# Autodesk Inventor assembly: Bucket+Magnets
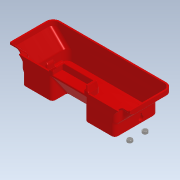
[picture p0: Inventor's stored thumbnail of the model, 180x180]
Saved by Autodesk Inventor 2022.1 (Build 261234020, 234B)
## iProperties
Created: 2022-07-24
Part Number: Bucket+Magnets
Document SubType Name: Assembly
Designer: Rama
Author: Rama
## Documents named in this file (3)
- C:\Users\Rama\Desktop\GitHub\Voron-2-Mods\Mandalaroseworks\BedPan\CAD\SRC\Manual_Helpers\Bucket+Magnets.iam
- C:\Users\Rama\Desktop\GitHub\Voron-2-Mods\Mandalaroseworks\BedPan\CAD\SRC\Bucket\Bucket_Offset.iam
- C:\Users\Rama\Desktop\RAMA_SBNG\ToolheadNEW\6x3 Magnet.ipt
## Components (5 placed, 2 different names)
1. Bucket_Offset:1 [sub-assembly]
2. 6x3 Magnet:1
3. 6x3 Magnet:2
4. 6x3 Magnet:3
5. 6x3 Magnet:4
## Relationships (7: Mate 4, Flush 3)
- [Flush]: 6x3 Magnet:2 ↔ 6x3 Magnet:3
- [Flush]: 6x3 Magnet:1 ↔ 6x3 Magnet:4
- [Flush]: 6x3 Magnet:3 ↔ 6x3 Magnet:4
- [Mate]: Bucket_Offset:1 ↔ 6x3 Magnet:2
- [Mate]: Bucket_Offset:1 ↔ 6x3 Magnet:3
- [Mate]: Bucket_Offset:1 ↔ 6x3 Magnet:1
- [Mate]: Bucket_Offset:1 ↔ 6x3 Magnet:4
